# Autodesk Inventor assembly: gearbox_version1
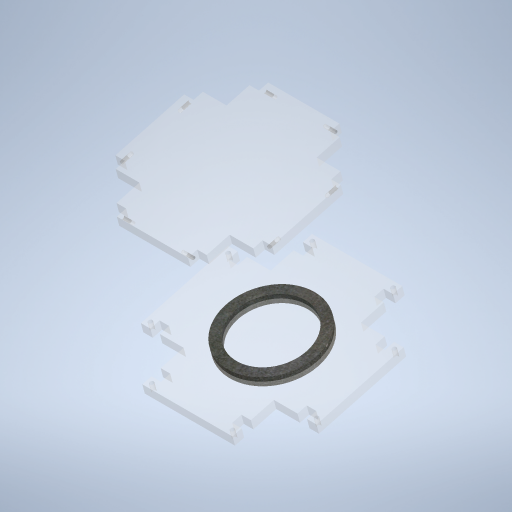
[picture p0: Inventor's stored thumbnail of the model, 512x512]
Saved by Autodesk Inventor 2023 (Build 270158000, 158)
## iProperties
Created: 2023-07-07
Part Number: gearbox_version1
Description: STEP AP203
Document SubType Name: Assembly
Designer: 310611102
Mass: 7892.17 g
Surface Area: 5738.97 cm^2
Volume: 1948.18 cm^3
Density: 4.05104 g/cm^3
Sending System: SolidWorks 2019
Preprocessor: SwSTEP 2.0
Title: gearbox_version1.STEP
Revision Number: ANY
## Documents named in this file (24)
- C:\Users\310611102\Documents\Inventor\SSR\avionics_2023ver\actuator_system\gearbox_ver2\gearbox_version2.iam
- C:\Users\310611102\Documents\Inventor\SSR\avionics_2023ver\actuator_system\gearbox_ver2\gearbox_side.ipt
- C:\Users\310611102\Documents\Inventor\SSR\avionics_2023ver\actuator_system\gearbox_ver2\lower_side_gear.ipt
- C:\Users\310611102\Documents\Inventor\SSR\avionics_2023ver\actuator_system\gearbox_ver2\main_bevel_gear.ipt
- C:\Users\310611102\Documents\Inventor\SSR\avionics_2023ver\actuator_system\gearbox_ver2\side_bevel_gear.ipt
- C:\Users\310611102\Documents\Inventor\SSR\avionics_2023ver\actuator_system\gearbox_ver2\upper_side_gear.ipt
- C:\Users\310611102\Documents\Inventor\SSR\avionics_2023ver\actuator_system\gearbox_ver2\lower_screw.ipt
- C:\Users\310611102\Documents\Inventor\SSR\avionics_2023ver\actuator_system\gearbox_ver2\lower_bearing.ipt
- C:\Users\310611102\Documents\Inventor\SSR\avionics_2023ver\actuator_system\gearbox_ver2\3mm_gasket.ipt
- C:\Users\310611102\Documents\Inventor\SSR\avionics_2023ver\actuator_system\gearbox_ver2\m3screw.ipt
- C:\Users\310611102\Documents\Inventor\SSR\avionics_2023ver\actuator_system\gearbox_ver2\m3nut_2.4.ipt
- C:\Users\310611102\Documents\Inventor\SSR\avionics_2023ver\actuator_system\gearbox_ver2\7mm_gasket.ipt
- C:\Users\310611102\Documents\Inventor\SSR\avionics_2023ver\actuator_system\gearbox_ver2\upper_screw.ipt
- C:\Users\310611102\Documents\Inventor\SSR\avionics_2023ver\actuator_system\gearbox_ver2\upper_3mm_screw.ipt
- C:\Users\310611102\Documents\Inventor\SSR\avionics_2023ver\actuator_system\gearbox_ver2\upper_bearing.ipt
- C:\Users\310611102\Documents\Inventor\SSR\avionics_2023ver\actuator_system\gearbox_ver2\main_bearing.ipt
- C:\Users\310611102\Documents\Inventor\SSR\avionics_2023ver\actuator_system\gearbox_ver2\gearbox_base.ipt
- C:\Users\310611102\Documents\Inventor\SSR\avionics_2023ver\actuator_system\gearbox_ver2\gearbox_cap.ipt
- C:\Users\310611102\Documents\Inventor\SSR\avionics_2023ver\actuator_system\gearbox_ver2\m7lower_screw.ipt
- C:\Users\310611102\Documents\Inventor\SSR\avionics_2023ver\actuator_system\gearbox_ver2\7mm_nut.ipt
- C:\Users\310611102\Documents\Inventor\SSR\avionics_2023ver\actuator_system\gearbox_ver2\m7lower_screw_MIR1.ipt
- C:\Users\310611102\Documents\Inventor\SSR\avionics_2023ver\actuator_system\gearbox_ver2\7mm_nut_MIR1.ipt
- C:\Users\310611102\Documents\Inventor\SSR\avionics_2023ver\actuator_system\gearbox_ver2\m7lower_screw_MIR2.ipt
- C:\Users\310611102\Documents\Inventor\SSR\avionics_2023ver\actuator_system\gearbox_ver2\7mm_nut_MIR2.ipt
## Components (124 placed, 45 different names)
1. main_bevel_gear_3
2. main_bearing_34
3. gearbox_base_35 — Mate:2, Flush:1, Mate:3
4. gearbox_cap:1 — Mate:4, Flush:2, Flush:3
5. 7mm_gasket_37
6. lower_side_gear_43
7. side_bevel_gear_46
8. m3screw_49
9. m3screw_52
10. 3mm_gasket_55
11. m3nut_2.4_58
12. 7mm_gasket_61
13. 3mm_gasket_70
14. m3nut_2.4_73
15. 7mm_gasket_76
16. 3mm_gasket_82
17. m3nut_2.4_85
18. 7mm_gasket_91
19. gearbox_side_94 — Mate:2, Flush:1, Mate:3, Mate:4, Flush:2, Flush:3
20. upper_3mm_screw_97
21. upper_3mm_screw_100
22. upper_side_gear_103
23. lower_bearing_109
24. lower_screw_112
25. upper_bearing_121
26. upper_screw_124
27. 7mm_nut_MIR2:1
28. m7lower_screw_MIR2:1
29. 7mm_nut:2 — Insert:4
30. m7lower_screw:2 — Insert:3
31. 7mm_nut_MIR1:1
32. m7lower_screw_MIR1:1
33. m7lower_screw:1 — Insert:1
34. 7mm_nut:1 — Insert:2
35. 7mm_gasket:15
36. lower_side_gear:3
37. side_bevel_gear:3
38. m3screw:7
39. m3screw:8
40. 3mm_gasket:12
41. m3nut_2.4:12
42. 7mm_gasket:16
43. 3mm_gasket:13
44. m3nut_2.4:13
45. 7mm_gasket:17
46. 3mm_gasket:14
47. m3nut_2.4:14
48. 7mm_gasket:18
49. gearbox_side:3
50. upper_3mm_screw:7
51. upper_3mm_screw:8
52. upper_side_gear:3
53. lower_bearing:3
54. lower_screw:3
55. upper_bearing:3
56. upper_screw:3
57. 7mm_nut_MIR2:2
58. m7lower_screw_MIR2:2
59. 7mm_nut:3
60. m7lower_screw:3
61. 7mm_nut_MIR1:2
62. m7lower_screw_MIR1:2
63. m7lower_screw:6
64. 7mm_nut:6
65. 7mm_gasket:19
66. lower_side_gear:4
67. side_bevel_gear:4
68. m3screw:9
69. m3screw:10
70. 3mm_gasket:15
71. m3nut_2.4:15
72. 7mm_gasket:20
73. 3mm_gasket:16
74. m3nut_2.4:16
75. 7mm_gasket:21
76. 3mm_gasket:17
77. m3nut_2.4:17
78. 7mm_gasket:22
79. gearbox_side:4
80. upper_3mm_screw:9
81. upper_3mm_screw:10
82. upper_side_gear:4
83. lower_bearing:4
84. lower_screw:4
85. upper_bearing:4
86. upper_screw:4
87. 7mm_nut_MIR2:3
88. m7lower_screw_MIR2:3
89. 7mm_nut:4
90. m7lower_screw:4
91. 7mm_nut_MIR1:3
92. m7lower_screw_MIR1:3
93. m7lower_screw:7
94. 7mm_nut:7
95. 7mm_gasket:23 — Insert:1
96. lower_side_gear:5
97. side_bevel_gear:5
98. m3screw:11
99. m3screw:12
100. 3mm_gasket:18
101. m3nut_2.4:18
102. 7mm_gasket:24
103. 3mm_gasket:19
104. m3nut_2.4:19
105. 7mm_gasket:25
106. 3mm_gasket:20
107. m3nut_2.4:20
108. 7mm_gasket:26 — Insert:3
109. gearbox_side:5
110. upper_3mm_screw:11
111. upper_3mm_screw:12
112. upper_side_gear:5
113. lower_bearing:5 — Insert:2
114. lower_screw:5
115. upper_bearing:5 — Insert:4
116. upper_screw:5
117. 7mm_nut_MIR2:4
118. m7lower_screw_MIR2:4
119. 7mm_nut:5
120. m7lower_screw:5
121. 7mm_nut_MIR1:4
122. m7lower_screw_MIR1:4
123. m7lower_screw:8
124. 7mm_nut:8
## Component patterns: (4 elements, first: 7mm_gasket_37 + lower_side_gear_43 + side_bevel_gear_46 + m3screw_49 + m3screw_52 + 3mm_gasket_55 + m3nut_2.4_58 + 7mm_gasket_61 + 3mm_gasket_70 + m3nut_2.4_73 + 7mm_gasket_76 + 3mm_gasket_82 + m3nut_2.4_85 + 7mm_gasket_91 + gearbox_side_94 + upper_3mm_screw_97 + upper_3mm_screw_100 + upper_side_gear_103 + lower_bearing_109 + lower_screw_112 + upper_bearing_121 + upper_screw_124 + 7mm_nut_MIR2:1 + m7lower_screw_MIR2:1 + 7mm_nut:2 + m7lower_screw:2 + 7mm_nut_MIR1:1 + m7lower_screw_MIR1:1 + m7lower_screw:1 + 7mm_nut:1)
## Relationships (10: Insert 4, Mate 3, Flush 3)
- Mate:2: gearbox_base_35 ↔ gearbox_side_94
- Flush:1: gearbox_base_35 ↔ gearbox_side_94
- Mate:3: gearbox_base_35 ↔ gearbox_side_94
- Mate:4: gearbox_cap:1 ↔ gearbox_side_94
- Flush:2: gearbox_cap:1 ↔ gearbox_side_94
- Flush:3: gearbox_cap:1 ↔ gearbox_side_94
- Insert:1: m7lower_screw:1 ↔ 7mm_gasket:23
- Insert:2: 7mm_nut:1 ↔ lower_bearing:5
- Insert:3: m7lower_screw:2 ↔ 7mm_gasket:26
- Insert:4: 7mm_nut:2 ↔ upper_bearing:5
